# Autodesk Inventor assembly: assemblage_robot
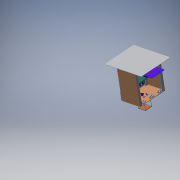
[picture p0: Inventor's stored thumbnail of the model, 180x180]
Saved by Autodesk Inventor 2017 (Build 210142000, 142)
## iProperties
Created: 2017-04-14
Part Number: assemblage_robot
Document SubType Name: Assembly
Designer: franc
Author: franc
## Documents named in this file (22)
- C:\Users\franc\Desktop\EsialRobotik\Mecanique\2017\robot-2017\assemblage_robot.iam
- C:\Users\franc\Desktop\EsialRobotik\Mecanique\2017\robot-2017\base_robot.ipt
- C:\Users\franc\Desktop\EsialRobotik\Mecanique\2017\base roulante\assemblage_base_amovible.iam
- C:\Users\franc\Desktop\EsialRobotik\Mecanique\2017\robot-2017\profile_alu.ipt
- C:\Users\franc\Desktop\EsialRobotik\Mecanique\2017\robot-2017\equerre_basse.ipt
- C:\Users\franc\Desktop\EsialRobotik\Mecanique\2017\robot-2017\equerre_haute.ipt
- C:\Users\franc\Desktop\EsialRobotik\Mecanique\2017\robot-2017\etage_support_minerai.ipt
- C:\Users\franc\Desktop\EsialRobotik\Mecanique\2017\robot-2017\AX12-minerai\ax12_wheel.ipt
- C:\Users\franc\Desktop\EsialRobotik\Mecanique\2017\robot-2017\AX12-minerai\ax12_box.ipt
- C:\Users\franc\Desktop\EsialRobotik\Mecanique\2017\robot-2017\AX12-minerai\ax12_cog.ipt
- C:\Users\franc\Desktop\EsialRobotik\Mecanique\2017\robot-2017\AX12-minerai\plaque.ipt
- C:\Users\franc\Desktop\EsialRobotik\Mecanique\2017\robot-2017\AX12-minerai\F2.ipt
- C:\Users\franc\Desktop\EsialRobotik\Mecanique\2017\robot-2017\AX12-minerai\F3.ipt
- C:\Users\franc\Desktop\EsialRobotik\Mecanique\2017\robot-2017\face_lateral_robot.ipt
- C:\Users\franc\Desktop\EsialRobotik\Mecanique\2017\robot-2017\module_lunaire.ipt
- C:\Users\franc\Desktop\EsialRobotik\Mecanique\2017\robot-2017\pince\pince.iam
- C:\Users\franc\Desktop\EsialRobotik\Mecanique\2017\robot-2017\toit_robot.ipt
- C:\Users\franc\Desktop\EsialRobotik\Mecanique\composants\RPlidar-A2M4\RPLIDAR A2.iam
- C:\Users\franc\Desktop\EsialRobotik\Mecanique\2017\robot-2017\support_balise.ipt
- C:\Users\franc\Desktop\EsialRobotik\Mecanique\2017\robot-2017\mat_support_balise.ipt
- C:\Users\franc\Desktop\EsialRobotik\Mecanique\2017\robot-2017\support_arriere.iam
- C:\Users\franc\Desktop\EsialRobotik\Mecanique\composants\SRF04\SRF04_sur_support.iam
## Components (37 placed, 21 different names)
1. base_robot:1 — Mate:1, Mate:2, Mate:3, Mate:12, Flush:7, Mate:14, Mate:15, Mate:17, Mate:20, Flush:12, Mate:24, Mate:31, Mate:33, Mate:35, Mate:36, Mate:37, Mate:40, Mate:41, Mate:43, Mate:44, Mate:46, Mate:47, Mate:50, Mate:51, Flush:13, Mate:52, Mate:73, Mate:75, Mate:78, Mate:79, Mate:80
2. assemblage_base_amovible:1 [sub-assembly] — Mate:1, Mate:2, Mate:3, Mate:102
3. profile_alu:1 — Mate:24, Mate:42, Mate:53, Mate:71, Mate:74, Flush:16, Mate:77
4. profile_alu:2 — Mate:20, Flush:12, Mate:45, Mate:49, Mate:72, Mate:93
5. profile_alu:3 — Mate:12, Flush:7, Mate:34, Mate:38, Mate:69
6. profile_alu:4 — Mate:17, Mate:30, Mate:32, Flush:13, Mate:67, Flush:14, Flush:15, Mate:76
7. equerre_basse:1 — Mate:14, Mate:15, Mate:67, Mate:76
8. equerre_haute:1 — Mate:30, Mate:31, Mate:32, Mate:52
9. equerre_basse:2 — Mate:33, Mate:34, Mate:35
10. equerre_haute:2 — Mate:36, Mate:37, Mate:38
11. equerre_basse:3 — Mate:40, Mate:41, Mate:71, Mate:77
12. equerre_haute:3 — Mate:42, Mate:43, Mate:44, Mate:53
13. equerre_basse:4 — Mate:45, Mate:46, Mate:47
14. equerre_haute:4 — Mate:49, Mate:50, Mate:51
15. etage_support_minerai:1 — Mate:64, Mate:65, Mate:66, Mate:69, Flush:14
16. ax12_wheel:1
17. ax12_box:1
18. ax12_cog:1
19. plaque:1 — Mate:102
20. F2:1
21. F3:1 — Mate:64, Mate:65, Mate:66
22. face_lateral_robot:1 — Mate:72, Flush:15, Mate:73
23. face_lateral_robot:2 — Mate:74, Flush:16, Mate:75, Flush:17, Flush:18, Mate:86, Flush:24
24. module_lunaire:1 — Mate:81, Mate:82
25. pince:1 [sub-assembly] — Mate:78, Mate:79, Mate:80, Mate:81, Mate:82
26. toit_robot:1 — Mate:83, Mate:84, Mate:85, Flush:17, Flush:18, Mate:86, Mate:87, Mate:88, Mate:89, Flush:20, Mate:90, Mate:91, Mate:92, Flush:25, Mate:94, Mate:95, Mate:96, Mate:97, Mate:98, Mate:99, Mate:100, Mate:101
27. RPLIDAR A2:1 [sub-assembly] — Mate:83, Mate:84, Mate:85
28. support_balise:1 — Mate:87, Mate:88, Flush:19, Flush:21, Flush:22, Flush:23
29. mat_support_balise:1 — Mate:90, Flush:21
30. mat_support_balise:2 — Mate:91, Flush:22
31. mat_support_balise:3 — Mate:92, Flush:23
32. mat_support_balise:4 — Mate:89, Flush:19, Flush:20
33. support_arriere:1 [sub-assembly] — Mate:93, Flush:24, Flush:25
34. SRF04_sur_support:1 [sub-assembly] — Mate:96, Mate:99
35. SRF04_sur_support:2 [sub-assembly] — Mate:95, Mate:97
36. SRF04_sur_support:3 [sub-assembly] — Mate:94, Mate:98
37. SRF04_sur_support:4 [sub-assembly] — Mate:100, Mate:101
## Relationships (93: Mate 77, Flush 15, Insert 1)
- Mate:1: base_robot:1 ↔ assemblage_base_amovible:1
- Mate:2: base_robot:1 ↔ assemblage_base_amovible:1
- Mate:3: base_robot:1 ↔ assemblage_base_amovible:1
- Mate:12: base_robot:1 ↔ profile_alu:3
- Flush:7: base_robot:1 ↔ profile_alu:3
- Mate:14: base_robot:1 ↔ equerre_basse:1
- Mate:15: base_robot:1 ↔ equerre_basse:1
- Mate:17: base_robot:1 ↔ profile_alu:4
- Mate:20: base_robot:1 ↔ profile_alu:2
- Flush:12: base_robot:1 ↔ profile_alu:2
- Mate:24: base_robot:1 ↔ profile_alu:1
- Mate:30: profile_alu:4 ↔ equerre_haute:1
- Mate:31: base_robot:1 ↔ equerre_haute:1
- Mate:32: profile_alu:4 ↔ equerre_haute:1
- Mate:33: base_robot:1 ↔ equerre_basse:2
- Mate:34: profile_alu:3 ↔ equerre_basse:2
- Mate:35: base_robot:1 ↔ equerre_basse:2
- Mate:36: base_robot:1 ↔ equerre_haute:2
- Mate:37: base_robot:1 ↔ equerre_haute:2
- Mate:38: profile_alu:3 ↔ equerre_haute:2
- Mate:40: base_robot:1 ↔ equerre_basse:3
- Mate:41: base_robot:1 ↔ equerre_basse:3
- Mate:42: profile_alu:1 ↔ equerre_haute:3
- Mate:43: base_robot:1 ↔ equerre_haute:3
- Mate:44: base_robot:1 ↔ equerre_haute:3
- Mate:45: profile_alu:2 ↔ equerre_basse:4
- Mate:46: base_robot:1 ↔ equerre_basse:4
- Mate:47: base_robot:1 ↔ equerre_basse:4
- Mate:49: profile_alu:2 ↔ equerre_haute:4
- Mate:50: base_robot:1 ↔ equerre_haute:4
- Mate:51: base_robot:1 ↔ equerre_haute:4
- Flush:13 (5 mm): base_robot:1 ↔ profile_alu:4
- Mate:52: base_robot:1 ↔ equerre_haute:1
- Mate:53: profile_alu:1 ↔ equerre_haute:3
- [Insert]: ax12_wheel:1 ↔ ax12_box:1
- [Mate]: ax12_wheel:1 ↔ F2:1
- [Mate]: ax12_wheel:1 ↔ F2:1
- [Mate]: ax12_wheel:1 ↔ F2:1
- [Mate]: plaque:1 ↔ F2:1
- [Mate]: plaque:1 ↔ F2:1
- [Mate]: plaque:1 ↔ F2:1
- [Mate]: ax12_box:1 ↔ F3:1
- [Mate]: ax12_box:1 ↔ F3:1
- [Mate]: ax12_box:1 ↔ F3:1
- Mate:64: etage_support_minerai:1 ↔ F3:1
- Mate:65: etage_support_minerai:1 ↔ F3:1
- Mate:66: etage_support_minerai:1 ↔ F3:1
- Mate:67: profile_alu:4 ↔ equerre_basse:1
- Mate:69: profile_alu:3 ↔ etage_support_minerai:1
- Flush:14: profile_alu:4 ↔ etage_support_minerai:1
- Mate:71: profile_alu:1 ↔ equerre_basse:3
- Mate:72: profile_alu:2 ↔ face_lateral_robot:1
- Flush:15: profile_alu:4 ↔ face_lateral_robot:1
- Mate:73: base_robot:1 ↔ face_lateral_robot:1
- Mate:74: profile_alu:1 ↔ face_lateral_robot:2
- Flush:16: profile_alu:1 ↔ face_lateral_robot:2
- Mate:75: base_robot:1 ↔ face_lateral_robot:2
- Mate:76: profile_alu:4 ↔ equerre_basse:1
- Mate:77: profile_alu:1 ↔ equerre_basse:3
- Mate:78: base_robot:1 ↔ pince:1
- Mate:79: base_robot:1 ↔ pince:1
- Mate:80: base_robot:1 ↔ pince:1
- Mate:81: module_lunaire:1 ↔ pince:1
- Mate:82: module_lunaire:1 ↔ pince:1
- Mate:83: toit_robot:1 ↔ RPLIDAR A2:1
- Mate:84: toit_robot:1 ↔ RPLIDAR A2:1
- Mate:85: toit_robot:1 ↔ RPLIDAR A2:1
- Flush:17: face_lateral_robot:2 ↔ toit_robot:1
- Flush:18: face_lateral_robot:2 ↔ toit_robot:1
- Mate:86: face_lateral_robot:2 ↔ toit_robot:1
- Mate:87: toit_robot:1 ↔ support_balise:1
- Mate:88: toit_robot:1 ↔ support_balise:1
- Mate:89: toit_robot:1 ↔ mat_support_balise:4
- Flush:19: support_balise:1 ↔ mat_support_balise:4
- Flush:20: toit_robot:1 ↔ mat_support_balise:4
- Mate:90: toit_robot:1 ↔ mat_support_balise:1
- Flush:21: support_balise:1 ↔ mat_support_balise:1
- Mate:91: toit_robot:1 ↔ mat_support_balise:2
- Flush:22: support_balise:1 ↔ mat_support_balise:2
- Mate:92: toit_robot:1 ↔ mat_support_balise:3
- Flush:23: support_balise:1 ↔ mat_support_balise:3
- Mate:93: profile_alu:2 ↔ support_arriere:1
- Flush:24: face_lateral_robot:2 ↔ support_arriere:1
- Flush:25: toit_robot:1 ↔ support_arriere:1
- Mate:94: toit_robot:1 ↔ SRF04_sur_support:3
- Mate:95: toit_robot:1 ↔ SRF04_sur_support:2
- Mate:96: toit_robot:1 ↔ SRF04_sur_support:1
- Mate:97: toit_robot:1 ↔ SRF04_sur_support:2
- Mate:98: toit_robot:1 ↔ SRF04_sur_support:3
- Mate:99: toit_robot:1 ↔ SRF04_sur_support:1
- Mate:100: toit_robot:1 ↔ SRF04_sur_support:4
- Mate:101: toit_robot:1 ↔ SRF04_sur_support:4
- Mate:102 (60 mm): assemblage_base_amovible:1 ↔ plaque:1
## Named parameters: d80_d25 = 0 mm, d83_d28 = 0 mm, d88_d24 = 0 mm
